# Autodesk Inventor assembly: Little correction needed
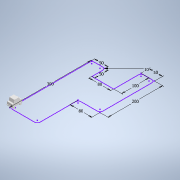
[picture p0: Inventor's stored thumbnail of the model, 180x180]
Saved by Autodesk Inventor 2021 (Build 250183000, 183)
## iProperties
Created: 2021-08-08
Part Number: Little correction needed
Document SubType Name: Assembly
Designer: Shammy Haider
Author: Shammy Haider
## Documents named in this file (3)
- D:\Designing\Autodesk inventor\Track car\Little correction needed.iam
- D:\Designing\Autodesk inventor\Track car\path.ipt
- D:\Designing\Autodesk inventor\Track car\Car.ipt
## Components (2 placed, 2 different names)
1. path:1 — Mate:1, Mate:2, Mate:3, Mate:4, Mate:5
2. Car:1 — Mate:4, Angle:1, Mate:5
## Relationships (6: Mate 5, Angle 1)
- Mate:1: path:1
- Mate:2: path:1
- Mate:3: path:1
- Mate:4: path:1 ↔ Car:1
- Angle:1 (0 deg): Car:1
- Mate:5: path:1 ↔ Car:1
